# Autodesk Inventor assembly: raspberry pi display
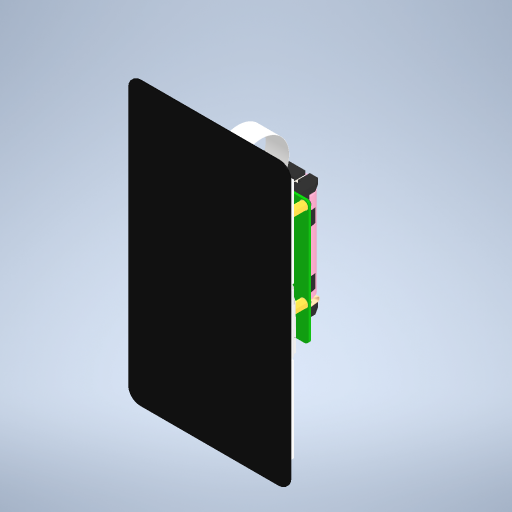
[picture p0: Inventor's stored thumbnail of the model, 512x512]
Saved by Autodesk Inventor 2023 (Build 270158000, 158)
## iProperties
Created: 2018-03-27
Part Number: raspberry pi display
Document SubType Name: Assembly
Designer: tdal0
Sending System: Autodesk Inventor 2017
Preprocessor: ST-DEVELOPER v16.5
Title: C:\Users\moroz\Desktop\projects\SLS\корпус свой вариант\v3\электроника\raspberry pi display.stp
Author: moroz
## Documents named in this file (9)
- C:\4806\front panel parts\raspberry pi display.iam
- C:\4806\front panel parts\raspberry pi display.ipt
- C:\4806\front panel parts\Raspberry Pi 3 .ipt
- C:\4806\front panel parts\raspberry pi display module.ipt
- C:\4806\front panel parts\12mmgold.ipt
- C:\4806\front panel parts\cables.ipt
- C:\4806\front panel parts\ISO 7045 - M2,5 x 3 - 4.8 - H - ISO.ipt
- C:\4806\front panel parts\Hold_18650-2p_smd.iam
- C:\4806\front panel parts\20mmgold.ipt
## Components (17 placed, 8 different names)
1. raspberry pi display:1 — Mate:9, Mate:10, Mate:11, Mate:12, Mate:13
2. Raspberry Pi 3 :1 — Mate:40, Mate:42, Mate:43, Mate:44
3. raspberry pi display module:1 — Mate:1, Mate:2, Mate:3, Mate:4, Mate:5, Mate:6, Mate:7, Mate:8, Mate:13
4. стойка 12мм:1 — Mate:3, Mate:4, Mate:10, Mate:35
5. стойка 12мм:2 — Mate:5, Mate:6, Mate:11, Mate:37, Mate:44
6. стойка 12мм:3 — Mate:1, Mate:2, Mate:9, Mate:33
7. стойка 12мм:4 — Mate:7, Mate:8, Mate:12, Mate:39
8. cables:1
9. ISO 7045 H M2,5 x 3 - 4.8 - H:1 — Mate:27, Mate:28, Mate:46
10. ISO 7045 H M2,5 x 3 - 4.8 - H:2 — Mate:29, Mate:32
11. ISO 7045 H M2,5 x 3 - 4.8 - H:3 — Mate:30, Mate:31, Mate:45
12. ISO 7045 H M2,5 x 3 - 4.8 - H:4 — Mate:25, Mate:26
13. Hold_18650-2p_smd:1 [sub-assembly] — Mate:25, Mate:26, Mate:27, Mate:28, Mate:29, Mate:30, Mate:31, Mate:32, Mate:34, Mate:36, Mate:38, Mate:41
14. 20mmgold:1 — Mate:37, Mate:38, Mate:42, Mate:45
15. 20mmgold:2 — Mate:39, Mate:40, Mate:41
16. 20mmgold:3 — Mate:35, Mate:36
17. 20mmgold:4 — Mate:33, Mate:34, Mate:43, Mate:46
## Relationships (35: Mate 35)
- Mate:1: raspberry pi display module:1 ↔ стойка 12мм:3
- Mate:2: raspberry pi display module:1 ↔ стойка 12мм:3
- Mate:3: raspberry pi display module:1 ↔ стойка 12мм:1
- Mate:4: raspberry pi display module:1 ↔ стойка 12мм:1
- Mate:5: raspberry pi display module:1 ↔ стойка 12мм:2
- Mate:6: raspberry pi display module:1 ↔ стойка 12мм:2
- Mate:7: raspberry pi display module:1 ↔ стойка 12мм:4
- Mate:8: raspberry pi display module:1 ↔ стойка 12мм:4
- Mate:9: raspberry pi display:1 ↔ стойка 12мм:3
- Mate:10: raspberry pi display:1 ↔ стойка 12мм:1
- Mate:11: raspberry pi display:1 ↔ стойка 12мм:2
- Mate:12: raspberry pi display:1 ↔ стойка 12мм:4
- Mate:13: raspberry pi display:1 ↔ raspberry pi display module:1
- Mate:25: ISO 7045 H M2,5 x 3 - 4.8 - H:4 ↔ Hold_18650-2p_smd:1
- Mate:26: ISO 7045 H M2,5 x 3 - 4.8 - H:4 ↔ Hold_18650-2p_smd:1
- Mate:27: ISO 7045 H M2,5 x 3 - 4.8 - H:1 ↔ Hold_18650-2p_smd:1
- Mate:28: ISO 7045 H M2,5 x 3 - 4.8 - H:1 ↔ Hold_18650-2p_smd:1
- Mate:29: ISO 7045 H M2,5 x 3 - 4.8 - H:2 ↔ Hold_18650-2p_smd:1
- Mate:30: ISO 7045 H M2,5 x 3 - 4.8 - H:3 ↔ Hold_18650-2p_smd:1
- Mate:31: ISO 7045 H M2,5 x 3 - 4.8 - H:3 ↔ Hold_18650-2p_smd:1
- Mate:32: ISO 7045 H M2,5 x 3 - 4.8 - H:2 ↔ Hold_18650-2p_smd:1
- Mate:33: стойка 12мм:3 ↔ 20mmgold:4
- Mate:34: Hold_18650-2p_smd:1 ↔ 20mmgold:4
- Mate:35: стойка 12мм:1 ↔ 20mmgold:3
- Mate:36: Hold_18650-2p_smd:1 ↔ 20mmgold:3
- Mate:37: стойка 12мм:2 ↔ 20mmgold:1
- Mate:38: Hold_18650-2p_smd:1 ↔ 20mmgold:1
- Mate:39: стойка 12мм:4 ↔ 20mmgold:2
- Mate:40: Raspberry Pi 3 :1 ↔ 20mmgold:2
- Mate:41: Hold_18650-2p_smd:1 ↔ 20mmgold:2
- Mate:42: Raspberry Pi 3 :1 ↔ 20mmgold:1
- Mate:43: Raspberry Pi 3 :1 ↔ 20mmgold:4
- Mate:44: Raspberry Pi 3 :1 ↔ стойка 12мм:2
- Mate:45: ISO 7045 H M2,5 x 3 - 4.8 - H:3 ↔ 20mmgold:1
- Mate:46: ISO 7045 H M2,5 x 3 - 4.8 - H:1 ↔ 20mmgold:4
